# Autodesk Inventor assembly: Assembly1
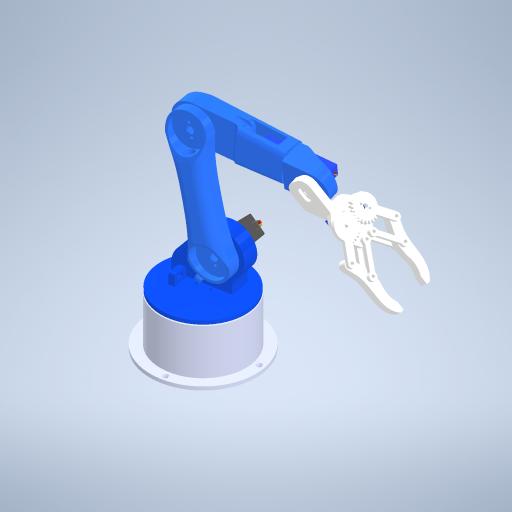
[picture p0: Inventor's stored thumbnail of the model, 512x512]
Saved by Autodesk Inventor 2024 (Build 280153000, 153)
## iProperties
Created: 2023-08-29
Part Number: Assembly1
Document SubType Name: Assembly
Designer: jebes windows
Author: jebes windows
## iProperties of the stored document Waist.ipt
Created: 2023-08-29
Part Number: Waist
Material: Generic
Document SubType Name: Modeling
Designer: jebes windows
Density: 1 g/cm^3
Appearance: Default
Author: jebes windows
Revision Number: ANY
## iProperties of the stored document gear1.ipt
Created: 2023-08-29
Part Number: gear1
Material: Generic
Document SubType Name: Modeling
Designer: jebes windows
Density: 1 g/cm^3
Appearance: Default
Author: jebes windows
Revision Number: ANY
## iProperties of the stored document Arm 01.ipt
Created: 2023-08-29
Part Number: Arm 01
Material: Generic
Document SubType Name: Modeling
Designer: jebes windows
Density: 1 g/cm^3
Appearance: Default
Author: jebes windows
Revision Number: ANY
## iProperties of the stored document Gripper Assembly.iam
Created: 2023-08-29
Part Number: Gripper Assembly
Document SubType Name: Assembly
Designer: jebes windows
Author: jebes windows
Revision Number: ANY
## iProperties of the stored document Arm 03.ipt
Created: 2023-08-29
Part Number: Arm 03
Material: Generic
Document SubType Name: Modeling
Designer: jebes windows
Density: 1 g/cm^3
Appearance: Default
Author: jebes windows
Revision Number: ANY
## iProperties of the stored document gear2.ipt
Created: 2023-08-29
Part Number: gear2
Material: Generic
Document SubType Name: Modeling
Designer: jebes windows
Density: 1 g/cm^3
Appearance: Default
Author: jebes windows
Revision Number: ANY
## iProperties of the stored document grip link 1.ipt
Created: 2023-08-29
Part Number: grip link 1
Material: Generic
Document SubType Name: Modeling
Designer: jebes windows
Density: 1 g/cm^3
Appearance: Default
Author: jebes windows
Revision Number: ANY
## iProperties of the stored document Servo Motor MG996R.ipt
Created: 2023-08-29
Part Number: Servo Motor MG996R
Material: Generic
Document SubType Name: Modeling
Designer: jebes windows
Density: 1 g/cm^3
Appearance: Default
Author: jebes windows
Revision Number: ANY
## iProperties of the stored document Robotic Arm 3D Model.iam
Created: 2021-12-01
Part Number: Robotic Arm 3D Model
Description: STEP AP214
Document SubType Name: Assembly
Designer: jebes windows
Sending System: SolidWorks 2022
Preprocessor: SwSTEP 2.0
Title: Robotic Arm 3D Model.STEP
Revision Number: ANY
## iProperties of the stored document Servo Motor Micro  9g.ipt
Created: 2023-08-29
Part Number: Servo Motor Micro  9g
Material: Generic
Document SubType Name: Modeling
Designer: jebes windows
Density: 1 g/cm^3
Appearance: Default
Author: jebes windows
Revision Number: ANY
## iProperties of the stored document Gripper 1.ipt
Created: 2023-08-29
Part Number: Gripper 1
Material: Generic
Document SubType Name: Modeling
Designer: jebes windows
Density: 1 g/cm^3
Appearance: Default
Author: jebes windows
Revision Number: ANY
## iProperties of the stored document Gripper base.ipt
Created: 2023-08-29
Part Number: Gripper base
Material: Generic
Document SubType Name: Modeling
Designer: jebes windows
Density: 1 g/cm^3
Appearance: Default
Author: jebes windows
Revision Number: ANY
## iProperties of the stored document Arm 02 v3.ipt
Created: 2023-08-29
Part Number: Arm 02 v3
Material: Generic
Document SubType Name: Modeling
Designer: jebes windows
Density: 1 g/cm^3
Appearance: Default
Author: jebes windows
Revision Number: ANY
## iProperties of the stored document Base.ipt
Created: 2023-08-29
Part Number: Base
Material: Generic
Document SubType Name: Modeling
Designer: jebes windows
Density: 1 g/cm^3
Appearance: Default
Author: jebes windows
Revision Number: ANY
## Documents named in this file (18)
- **C:\Users\jebes windows\Documents\Inventor\Robotska_roka\Assembly1.iam*LocalDocs*xAaaaarbaAaaaaaaaAaaaawtvDg*Waist.ipt
- **C:\Users\jebes windows\Documents\Inventor\Robotska_roka\Assembly1.iam*LocalDocs*xAaaaahaaAaaaaaaaAaaaq3b5Dh*gear1.ipt
- **C:\Users\jebes windows\Documents\Inventor\Robotska_roka\Assembly1.iam*LocalDocs*xAaaaafcaAaaaaaaaAaaaahq1Wb*Arm 01.ipt
- **C:\Users\jebes windows\Documents\Inventor\Robotska_roka\Assembly1.iam*LocalDocs*xAaaaandaAaaaaaaaAaaaat2cIb*Gripper Assembly.iam
- **C:\Users\jebes windows\Documents\Inventor\Robotska_roka\Assembly1.iam*LocalDocs*xAaaaatbaAaaaaaaaAaaaqr1xKb*gear2.ipt
- **C:\Users\jebes windows\Documents\Inventor\Robotska_roka\Assembly1.iam*LocalDocs*xAaaaasdaAaaaaaaaAaaaaxsjQh*grip link 1.ipt
- **C:\Users\jebes windows\Documents\Inventor\Robotska_roka\Assembly1.iam*LocalDocs*xAaaaqldaAaaaaaaaAaaaafp0Ff*Gripper base.ipt
- **C:\Users\jebes windows\Documents\Inventor\Robotska_roka\Assembly1.iam*LocalDocs*xAaaaqcdaAaaaaaaaAaaaq01rJh*Gripper 1.ipt
- **C:\Users\jebes windows\Documents\Inventor\Robotska_roka\Assembly1.iam*LocalDocs*xAaaaqgdaAaaaaaaaAaaaauw3Rg*Servo Motor Micro  9g.ipt
- **C:\Users\jebes windows\Documents\Inventor\Robotska_roka\Assembly1.iam*LocalDocs*xAaaaqbaaAaaaaaaaAaaaajzoIe*Arm 03.ipt
- **C:\Users\jebes windows\Documents\Inventor\Robotska_roka\Assembly1.iam*LocalDocs*xAaaaasaaAaaaaaaaAaaaad3wDa*Servo Motor MG996R.ipt
- **C:\Users\jebes windows\Documents\Inventor\Robotska_roka\Assembly1.iam*LocalDocs*xAaaaaxcaAaaaaaaaAaaaqgnkLa*Robotic Arm 3D Model.iam
- **C:\Users\jebes windows\Documents\Inventor\Robotska_roka\Assembly1.iam*LocalDocs*xAaaaqzaaAaaaaaaaAaaaal2lIh*Base.ipt
- **C:\Users\jebes windows\Documents\Inventor\Robotska_roka\Assembly1.iam*LocalDocs*xAaaaqldaAaaaaaaaAaaaa3wyMf*Arm 02 v3.ipt
- C:\Users\jebes windows\Documents\Inventor\Robotska_roka\Assembly1.iam
- C:\Users\jebes windows\Downloads\52mm_Omni_Wheel__2599926\files\52mm_roller\52mm_roller.ipt
- C:\Users\jebes windows\Downloads\52mm_Omni_Wheel__2599926\files\52mm_Main_Body\52mm_Main_Body.ipt
- C:\Users\jebes windows\Downloads\Robotic Arm 3D Model(1)\Robotic Arm 3D Model.STEP
## Components (10 placed, 3 different names)
1. Robotic Arm 3D Model:1 [sub-assembly]
2. 52mm_roller:1 — Rotational:1
3. 52mm_Main_Body:1 — Rotational:1, Rotational:2, Rotational:3, Rotational:4, Rotational:5, Rotational:6, Rotational:7, Rotational:8
4. 52mm_roller:3 — Rotational:7
5. 52mm_roller:4 — Rotational:8
6. 52mm_roller:5 — Rotational:6
7. 52mm_roller:6 — Rotational:5
8. 52mm_roller:7 — Rotational:4
9. 52mm_roller:8 — Rotational:3
10. 52mm_roller:9 — Rotational:2
## Relationships (8: RevoluteJoint 8)
- Rotational:1 [RevoluteJoint]: 52mm_roller:1 ↔ 52mm_Main_Body:1
- Rotational:2 [RevoluteJoint]: 52mm_Main_Body:1 ↔ 52mm_roller:9
- Rotational:3 [RevoluteJoint]: 52mm_Main_Body:1 ↔ 52mm_roller:8
- Rotational:4 [RevoluteJoint]: 52mm_Main_Body:1 ↔ 52mm_roller:7
- Rotational:5 [RevoluteJoint]: 52mm_Main_Body:1 ↔ 52mm_roller:6
- Rotational:6 [RevoluteJoint]: 52mm_Main_Body:1 ↔ 52mm_roller:5
- Rotational:7 [RevoluteJoint]: 52mm_Main_Body:1 ↔ 52mm_roller:3
- Rotational:8 [RevoluteJoint]: 52mm_Main_Body:1 ↔ 52mm_roller:4
